# Autodesk Inventor assembly: ChassisBase
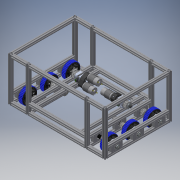
[picture p0: Inventor's stored thumbnail of the model, 180x180]
Saved by Autodesk Inventor 2018 (Build 220112000, 112)
## iProperties
Created: 2017-09-03
Part Number: ChassisBase
Document SubType Name: Assembly
Designer: snipe
Author: snipe
## Documents named in this file (13)
- E:\Clark\Assets\ClarkBodyV2.iam
- E:\Clark\Assets\pro20in.ipt
- E:\Clark\Assets\BearingBlock.ipt
- E:\Clark\Assets\DriveShaftA.iam
- E:\Clark\Assets\SideShaftA.iam
- E:\Clark\Assets\SideShaftB.iam
- E:\Clark\Assets\Profile_BaseModel_20mm\Profile_BaseModel_20mm-02.ipt
- E:\Clark\Assets\Profile_BaseModel_20mm.ipt
- E:\Clark\Assets\Profile_BaseModel_20mm\Profile_BaseModel_20mm-03.ipt
- E:\Clark\Assets\Profile_BaseModel_20mm\Profile_BaseModel_20mm-05.ipt
- E:\Clark\Assets\VPlan775dualinput.iam
- E:\Clark\Assets\24tPulley15mm.ipt
- E:\Clark\Assets\ShaftCollar.ipt
## Components (58 placed, 22 different names)
1. Profile_BaseModel_20mm-05:14 — Mate:142, Flush:135, Flush:136
2. Profile_BaseModel_20mm-05:13 — Mate:143, Flush:137, Flush:138
3. Profile_BaseModel_20mm-05:12 — Mate:137, Flush:129, Flush:130, Flush:131
4. Profile_BaseModel_20mm-05:11 — Mate:136, Flush:126, Flush:127, Flush:132
5. Profile_BaseModel_20mm-03:10 — Mate:133, Flush:120, Mate:134, Flush:121, Flush:122, Flush:123
6. Profile_BaseModel_20mm-03:9 — Mate:135, Flush:124, Flush:125
7. pro20in:1 — Mate:31, Flush:19, Mate:32, Mate:33, Flush:20, Flush:21, Mate:128, Flush:110, Flush:111, Mate:129, Flush:112, Flush:113
8. pro20in:2 — Mate:9, Flush:9, Mate:11, Flush:10, Flush:11, Mate:20, Flush:15, Mate:125, Flush:104, Flush:105, Flush:118, Mate:132, Flush:119
9. pro20in:3 — Flush:16, Mate:28, Flush:17, Mate:29, Flush:18, Mate:30, Mate:127, Flush:108, Flush:109, Mate:130, Flush:114, Flush:115
10. pro20in:4 — Mate:15, Mate:16, Flush:12, Flush:13, Flush:14, Mate:19, Flush:15, Mate:126, Flush:106, Flush:107, Mate:131, Flush:116, Flush:117
11. SideShaftA:1 [sub-assembly] — Mate:21, Mate:22, Mate:27, Mate:145, Mate:147, Mate:149
12. DriveShaftA:1 [sub-assembly] — Mate:23, Mate:24, Mate:140, Mate:147, Mate:148, Flush:149, Mate:173, Flush:184
13. SideShaftB:1 [sub-assembly] — Mate:25, Mate:26, Mate:141, Mate:148
14. SideShaftB:2 [sub-assembly] — Mate:88, Mate:93, Mate:144, Mate:149
15. DriveShaftA:2 [sub-assembly] — Mate:85, Mate:92, Mate:139, Mate:146, Flush:149, Mate:172, Flush:185
16. SideShaftA:2 [sub-assembly] — Mate:86, Mate:87, Mate:90, Mate:91, Mate:146
17. RightBack — Mate:11, Flush:11, Mate:141, Flush:143
18. RightCenter — Flush:10, Mate:20, Mate:140, Flush:144
19. RightFront — Mate:9, Flush:9, Mate:27, Mate:145, Flush:145, Mate:157
20. RightBack2 — Mate:16, Flush:14, Mate:17, Mate:25, Mate:26, Flush:141, Flush:143
21. RightCenter2 — Flush:12, Mate:17, Mate:18, Mate:19, Mate:23, Mate:24, Flush:140, Flush:144
22. RightFront2 — Mate:15, Flush:13, Mate:18, Mate:21, Mate:22, Flush:139, Flush:142, Flush:145, Mate:156
23. LeftBack — Mate:32, Flush:21, Mate:86, Mate:87, Mate:89, Flush:148
24. LeftCenter — Mate:31, Flush:19, Mate:35, Mate:85, Mate:89, Mate:92, Flush:147
25. LeftFront — Mate:33, Flush:20, Mate:35, Mate:88, Mate:93, Flush:146
26. LeftBack2 — Flush:18, Mate:30, Mate:90, Mate:91, Flush:141, Flush:148
27. LeftCenter2 — Flush:17, Mate:29, Mate:139, Flush:140, Flush:147
28. LeftFront2 — Flush:16, Mate:28, Flush:139, Mate:144, Flush:142, Flush:146
29. pro20in:9 — Mate:166, Flush:173, Mate:169, Flush:176, Mate:170
30. pro20in:10 — Mate:167, Flush:174, Mate:168, Flush:175, Mate:171
31. Profile_BaseModel_20mm-03:17 — Mate:165, Flush:166, Flush:167, Mate:166, Mate:167, Flush:174
32. Profile_BaseModel_20mm-03:18 — Mate:164, Flush:160, Flush:161
33. pro20in:5 — Mate:150, Flush:153, Mate:157
34. pro20in:6 — Mate:151, Flush:152, Mate:156, Flush:166, Mate:171
35. pro20in:7 — Mate:152, Flush:151, Flush:161, Flush:173, Mate:170
36. pro20in:8 — Mate:153, Flush:150
37. Profile_BaseModel_20mm-02:1 — Mate:125, Flush:104, Flush:105, Flush:132, Mate:138, Flush:133, Flush:134, Mate:182, Mate:183
38. Profile_BaseModel_20mm-02:2 — Mate:126, Flush:106, Flush:107, Mate:134, Flush:121, Flush:122, Mate:136, Flush:126, Flush:127, Mate:161, Flush:162, Flush:172
39. Profile_BaseModel_20mm-02:3 — Mate:127, Flush:108, Flush:109, Mate:133, Flush:120, Flush:123, Flush:131, Symmetry:7, Mate:158, Flush:154, Flush:155, Mate:164, Flush:158, Flush:160
40. Profile_BaseModel_20mm-02:4 — Mate:128, Flush:110, Flush:111, Mate:137, Flush:129, Flush:130, Mate:160, Flush:169
41. Profile_BaseModel_20mm-02:5 — Mate:129, Flush:112, Flush:113, Flush:138, Mate:153, Flush:150, Mate:163, Flush:170, Mate:180, Flush:186, Flush:187
42. Profile_BaseModel_20mm-02:6 — Mate:130, Flush:114, Flush:115, Mate:135, Flush:124, Flush:125, Mate:143, Flush:137, Symmetry:7, Mate:152, Flush:151, Mate:159, Flush:156, Flush:157, Mate:165, Flush:168
43. Profile_BaseModel_20mm-02:7 — Mate:131, Flush:116, Flush:117, Mate:142, Flush:135, Flush:136, Mate:151, Flush:152, Mate:162, Flush:165, Flush:167, Flush:171
44. Profile_BaseModel_20mm-02:8 — Flush:118, Mate:132, Flush:119, Mate:150, Flush:153, Mate:181, Flush:188, Flush:189
45. pro20in:11 — Mate:180, Flush:186, Flush:187
46. pro20in:12 — Mate:181, Flush:188, Flush:189, Mate:182, Mate:183
47. Profile_BaseModel_20mm-03:15 — Mate:158, Flush:154, Flush:155
48. Profile_BaseModel_20mm-03:16 — Mate:159, Flush:156, Flush:157
49. Profile_BaseModel_20mm-05:19 — Mate:160, Flush:158, Flush:169
50. Profile_BaseModel_20mm-05:20 — Mate:162, Flush:165, Flush:171
51. Profile_BaseModel_20mm-05:21 — Mate:161, Flush:162, Flush:172
52. Profile_BaseModel_20mm-05:22 — Mate:163, Flush:168, Flush:170
53. VPlan775dualinput:1 [sub-assembly] — Mate:169, Flush:176, Mate:172, Mate:178, Mate:179
54. VPlan775dualinput:2 [sub-assembly] — Mate:168, Flush:175, Mate:173, Mate:176, Mate:177
55. 24tPulley15mm:1 — Flush:177, Flush:178, Mate:176, Mate:177, Flush:184
56. ShaftCollar:1 — Flush:177, Flush:178
57. 24tPulley15mm:2 — Flush:182, Flush:183, Mate:178, Mate:179, Flush:185
58. ShaftCollar:2 — Flush:182, Flush:183
## Relationships (181: Flush 92, Mate 88, Symmetry 1)
- Mate:9: pro20in:2 ↔ RightFront
- Flush:9: pro20in:2 ↔ RightFront
- Mate:11: pro20in:2 ↔ RightBack
- Flush:10: pro20in:2 ↔ RightCenter
- Flush:11: pro20in:2 ↔ RightBack
- Mate:15: pro20in:4 ↔ RightFront2
- Mate:16: pro20in:4 ↔ RightBack2
- Flush:12: pro20in:4 ↔ RightCenter2
- Flush:13: pro20in:4 ↔ RightFront2
- Flush:14: pro20in:4 ↔ RightBack2
- Mate:17 (-147.447 mm): RightBack2 ↔ RightCenter2
- Mate:18 (147.447 mm): RightCenter2 ↔ RightFront2
- Mate:19: pro20in:4 ↔ RightCenter2
- Mate:20: pro20in:2 ↔ RightCenter
- Mate:21: SideShaftA:1 ↔ RightFront2
- Mate:22: SideShaftA:1 ↔ RightFront2
- Mate:23: DriveShaftA:1 ↔ RightCenter2
- Mate:24: DriveShaftA:1 ↔ RightCenter2
- Mate:25: SideShaftB:1 ↔ RightBack2
- Mate:26: SideShaftB:1 ↔ RightBack2
- Mate:27: SideShaftA:1 ↔ RightFront
- Flush:15: pro20in:2 ↔ pro20in:4
- Flush:16: pro20in:3 ↔ LeftFront2
- Mate:28: pro20in:3 ↔ LeftFront2
- Flush:17: pro20in:3 ↔ LeftCenter2
- Mate:29: pro20in:3 ↔ LeftCenter2
- Flush:18: pro20in:3 ↔ LeftBack2
- Mate:30: pro20in:3 ↔ LeftBack2
- Mate:31: pro20in:1 ↔ LeftCenter
- Flush:19: pro20in:1 ↔ LeftCenter
- Mate:32: pro20in:1 ↔ LeftBack
- Mate:33: pro20in:1 ↔ LeftFront
- Flush:20: pro20in:1 ↔ LeftFront
- Flush:21: pro20in:1 ↔ LeftBack
- Mate:35 (147.447 mm): LeftCenter ↔ LeftFront
- Mate:85: DriveShaftA:2 ↔ LeftCenter
- Mate:86: SideShaftA:2 ↔ LeftBack
- Mate:87: SideShaftA:2 ↔ LeftBack
- Mate:88: SideShaftB:2 ↔ LeftFront
- Mate:89 (147.447 mm): LeftBack ↔ LeftCenter
- Mate:90: SideShaftA:2 ↔ LeftBack2
- Mate:91: SideShaftA:2 ↔ LeftBack2
- Mate:92: DriveShaftA:2 ↔ LeftCenter
- Mate:93: SideShaftB:2 ↔ LeftFront
- Mate:125: pro20in:2 ↔ Profile_BaseModel_20mm-02:1
- Flush:104: pro20in:2 ↔ Profile_BaseModel_20mm-02:1
- Flush:105: pro20in:2 ↔ Profile_BaseModel_20mm-02:1
- Mate:126: pro20in:4 ↔ Profile_BaseModel_20mm-02:2
- Flush:106: pro20in:4 ↔ Profile_BaseModel_20mm-02:2
- Flush:107: pro20in:4 ↔ Profile_BaseModel_20mm-02:2
- Mate:127: pro20in:3 ↔ Profile_BaseModel_20mm-02:3
- Flush:108: pro20in:3 ↔ Profile_BaseModel_20mm-02:3
- Flush:109: pro20in:3 ↔ Profile_BaseModel_20mm-02:3
- Mate:128: pro20in:1 ↔ Profile_BaseModel_20mm-02:4
- Flush:110: pro20in:1 ↔ Profile_BaseModel_20mm-02:4
- Flush:111: pro20in:1 ↔ Profile_BaseModel_20mm-02:4
- Mate:129: pro20in:1 ↔ Profile_BaseModel_20mm-02:5
- Flush:112: pro20in:1 ↔ Profile_BaseModel_20mm-02:5
- Flush:113: pro20in:1 ↔ Profile_BaseModel_20mm-02:5
- Mate:130: pro20in:3 ↔ Profile_BaseModel_20mm-02:6
- Flush:114: pro20in:3 ↔ Profile_BaseModel_20mm-02:6
- Flush:115: pro20in:3 ↔ Profile_BaseModel_20mm-02:6
- Mate:131: pro20in:4 ↔ Profile_BaseModel_20mm-02:7
- Flush:116: pro20in:4 ↔ Profile_BaseModel_20mm-02:7
- Flush:117: pro20in:4 ↔ Profile_BaseModel_20mm-02:7
- Flush:118: pro20in:2 ↔ Profile_BaseModel_20mm-02:8
- Mate:132: pro20in:2 ↔ Profile_BaseModel_20mm-02:8
- Flush:119: pro20in:2 ↔ Profile_BaseModel_20mm-02:8
- Mate:133: Profile_BaseModel_20mm-03:10 ↔ Profile_BaseModel_20mm-02:3
- Flush:120: Profile_BaseModel_20mm-03:10 ↔ Profile_BaseModel_20mm-02:3
- Mate:134: Profile_BaseModel_20mm-03:10 ↔ Profile_BaseModel_20mm-02:2
- Flush:121: Profile_BaseModel_20mm-03:10 ↔ Profile_BaseModel_20mm-02:2
- Flush:122: Profile_BaseModel_20mm-03:10 ↔ Profile_BaseModel_20mm-02:2
- Flush:123: Profile_BaseModel_20mm-03:10 ↔ Profile_BaseModel_20mm-02:3
- Mate:135: Profile_BaseModel_20mm-03:9 ↔ Profile_BaseModel_20mm-02:6
- Flush:124: Profile_BaseModel_20mm-03:9 ↔ Profile_BaseModel_20mm-02:6
- Flush:125: Profile_BaseModel_20mm-03:9 ↔ Profile_BaseModel_20mm-02:6
- Mate:136: Profile_BaseModel_20mm-05:11 ↔ Profile_BaseModel_20mm-02:2
- Flush:126: Profile_BaseModel_20mm-05:11 ↔ Profile_BaseModel_20mm-02:2
- Flush:127: Profile_BaseModel_20mm-05:11 ↔ Profile_BaseModel_20mm-02:2
- Mate:137: Profile_BaseModel_20mm-05:12 ↔ Profile_BaseModel_20mm-02:4
- Flush:129: Profile_BaseModel_20mm-05:12 ↔ Profile_BaseModel_20mm-02:4
- Flush:130: Profile_BaseModel_20mm-05:12 ↔ Profile_BaseModel_20mm-02:4
- Flush:131: Profile_BaseModel_20mm-05:12 ↔ Profile_BaseModel_20mm-02:3
- Flush:132: Profile_BaseModel_20mm-05:11 ↔ Profile_BaseModel_20mm-02:1
- Mate:138: Profile_BaseModel_20mm-02:1
- Flush:133: Profile_BaseModel_20mm-02:1
- Flush:134: Profile_BaseModel_20mm-02:1
- Mate:139: DriveShaftA:2 ↔ LeftCenter2
- Mate:140: DriveShaftA:1 ↔ RightCenter
- Mate:141: SideShaftB:1 ↔ RightBack
- Mate:142: Profile_BaseModel_20mm-05:14 ↔ Profile_BaseModel_20mm-02:7
- Flush:135: Profile_BaseModel_20mm-05:14 ↔ Profile_BaseModel_20mm-02:7
- Flush:136: Profile_BaseModel_20mm-05:14 ↔ Profile_BaseModel_20mm-02:7
- Mate:143: Profile_BaseModel_20mm-05:13 ↔ Profile_BaseModel_20mm-02:6
- Flush:137: Profile_BaseModel_20mm-05:13 ↔ Profile_BaseModel_20mm-02:6
- Flush:138: Profile_BaseModel_20mm-05:13 ↔ Profile_BaseModel_20mm-02:5
- Flush:139: RightFront2 ↔ LeftFront2
- Symmetry:7: Profile_BaseModel_20mm-02:3 ↔ Profile_BaseModel_20mm-02:6
- Mate:144: SideShaftB:2 ↔ LeftFront2
- Mate:145: SideShaftA:1 ↔ RightFront
- Flush:140: RightCenter2 ↔ LeftCenter2
- Flush:141: RightBack2 ↔ LeftBack2
- Flush:142: RightFront2 ↔ LeftFront2
- Flush:143: RightBack ↔ RightBack2
- Flush:144: RightCenter ↔ RightCenter2
- Flush:145: RightFront ↔ RightFront2
- Flush:146: LeftFront ↔ LeftFront2
- Flush:147: LeftCenter ↔ LeftCenter2
- Flush:148: LeftBack ↔ LeftBack2
- Mate:146: DriveShaftA:2 ↔ SideShaftA:2
- Mate:147: SideShaftA:1 ↔ DriveShaftA:1
- Mate:148: DriveShaftA:1 ↔ SideShaftB:1
- Flush:149: DriveShaftA:1 ↔ DriveShaftA:2
- Mate:149: SideShaftA:1 ↔ SideShaftB:2
- Mate:150: pro20in:5 ↔ Profile_BaseModel_20mm-02:8
- Mate:151: pro20in:6 ↔ Profile_BaseModel_20mm-02:7
- Mate:152: pro20in:7 ↔ Profile_BaseModel_20mm-02:6
- Mate:153: pro20in:8 ↔ Profile_BaseModel_20mm-02:5
- Flush:150: pro20in:8 ↔ Profile_BaseModel_20mm-02:5
- Flush:151: pro20in:7 ↔ Profile_BaseModel_20mm-02:6
- Flush:152: pro20in:6 ↔ Profile_BaseModel_20mm-02:7
- Flush:153: pro20in:5 ↔ Profile_BaseModel_20mm-02:8
- Mate:156: RightFront2 ↔ pro20in:6
- Mate:157: RightFront ↔ pro20in:5
- Mate:158: Profile_BaseModel_20mm-02:3 ↔ Profile_BaseModel_20mm-03:15
- Flush:154: Profile_BaseModel_20mm-02:3 ↔ Profile_BaseModel_20mm-03:15
- Flush:155: Profile_BaseModel_20mm-02:3 ↔ Profile_BaseModel_20mm-03:15
- Mate:159: Profile_BaseModel_20mm-02:6 ↔ Profile_BaseModel_20mm-03:16
- Flush:156: Profile_BaseModel_20mm-02:6 ↔ Profile_BaseModel_20mm-03:16
- Flush:157: Profile_BaseModel_20mm-02:6 ↔ Profile_BaseModel_20mm-03:16
- Mate:160: Profile_BaseModel_20mm-02:4 ↔ Profile_BaseModel_20mm-05:19
- Mate:161: Profile_BaseModel_20mm-02:2 ↔ Profile_BaseModel_20mm-05:21
- Mate:162: Profile_BaseModel_20mm-02:7 ↔ Profile_BaseModel_20mm-05:20
- Mate:163: Profile_BaseModel_20mm-02:5 ↔ Profile_BaseModel_20mm-05:22
- Mate:164: Profile_BaseModel_20mm-03:18 ↔ Profile_BaseModel_20mm-02:3
- Mate:165: Profile_BaseModel_20mm-03:17 ↔ Profile_BaseModel_20mm-02:6
- Flush:158: Profile_BaseModel_20mm-02:3 ↔ Profile_BaseModel_20mm-05:19
- Flush:160: Profile_BaseModel_20mm-03:18 ↔ Profile_BaseModel_20mm-02:3
- Flush:161: Profile_BaseModel_20mm-03:18 ↔ pro20in:7
- Flush:162: Profile_BaseModel_20mm-02:2 ↔ Profile_BaseModel_20mm-05:21
- Flush:165: Profile_BaseModel_20mm-02:7 ↔ Profile_BaseModel_20mm-05:20
- Flush:166: Profile_BaseModel_20mm-03:17 ↔ pro20in:6
- Flush:167: Profile_BaseModel_20mm-03:17 ↔ Profile_BaseModel_20mm-02:7
- Flush:168: Profile_BaseModel_20mm-02:6 ↔ Profile_BaseModel_20mm-05:22
- Flush:169: Profile_BaseModel_20mm-02:4 ↔ Profile_BaseModel_20mm-05:19
- Flush:170: Profile_BaseModel_20mm-02:5 ↔ Profile_BaseModel_20mm-05:22
- Flush:171: Profile_BaseModel_20mm-02:7 ↔ Profile_BaseModel_20mm-05:20
- Flush:172: Profile_BaseModel_20mm-02:2 ↔ Profile_BaseModel_20mm-05:21
- Mate:166: pro20in:9 ↔ Profile_BaseModel_20mm-03:17
- Flush:173: pro20in:9 ↔ pro20in:7
- Mate:167: pro20in:10 ↔ Profile_BaseModel_20mm-03:17
- Flush:174: pro20in:10 ↔ Profile_BaseModel_20mm-03:17
- Mate:168: pro20in:10 ↔ VPlan775dualinput:2
- Flush:175: pro20in:10 ↔ VPlan775dualinput:2
- Mate:169: pro20in:9 ↔ VPlan775dualinput:1
- Flush:176: pro20in:9 ↔ VPlan775dualinput:1
- Mate:170 (26.9875 mm): pro20in:9 ↔ pro20in:7
- Mate:171 (26.9875 mm): pro20in:10 ↔ pro20in:6
- Mate:172 (97.409 mm): DriveShaftA:2 ↔ VPlan775dualinput:1
- Mate:173 (97.409 mm): DriveShaftA:1 ↔ VPlan775dualinput:2
- [Mate]: 24tPulley15mm:1 ↔ ShaftCollar:1
- [Mate]: 24tPulley15mm:2 ↔ ShaftCollar:2
- Flush:177: 24tPulley15mm:1 ↔ ShaftCollar:1
- Flush:178: 24tPulley15mm:1 ↔ ShaftCollar:1
- Mate:176: VPlan775dualinput:2 ↔ 24tPulley15mm:1
- Mate:177: VPlan775dualinput:2 ↔ 24tPulley15mm:1
- Flush:182: 24tPulley15mm:2 ↔ ShaftCollar:2
- Flush:183: 24tPulley15mm:2 ↔ ShaftCollar:2
- Mate:178: VPlan775dualinput:1 ↔ 24tPulley15mm:2
- Mate:179: VPlan775dualinput:1 ↔ 24tPulley15mm:2
- Flush:184: DriveShaftA:1 ↔ 24tPulley15mm:1
- Flush:185: DriveShaftA:2 ↔ 24tPulley15mm:2
- Mate:180: Profile_BaseModel_20mm-02:5 ↔ pro20in:11
- Flush:186: Profile_BaseModel_20mm-02:5 ↔ pro20in:11
- Flush:187: Profile_BaseModel_20mm-02:5 ↔ pro20in:11
- Mate:181: Profile_BaseModel_20mm-02:8 ↔ pro20in:12
- Flush:188: Profile_BaseModel_20mm-02:8 ↔ pro20in:12
- Flush:189: Profile_BaseModel_20mm-02:8 ↔ pro20in:12
- Mate:182: Profile_BaseModel_20mm-02:1 ↔ pro20in:12
- Mate:183: Profile_BaseModel_20mm-02:1 ↔ pro20in:12
## Named parameters: d478_d283 = 0 mm
